# Autodesk Inventor assembly: G20
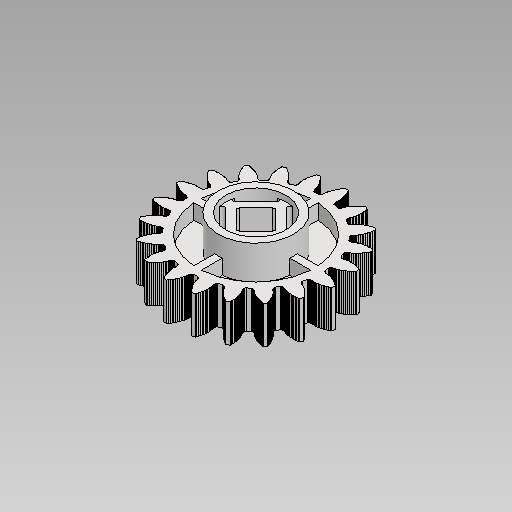
[picture p0: Inventor's stored thumbnail of the model, 512x512]
Saved by Autodesk Inventor 2020 (Build 240168000, 168)
## iProperties
Created: 2019-05-06
Part Number: G20
Document SubType Name: Assembly
Designer: Varga Daniel
Author: Varga Daniel
## Documents named in this file (3)
- C:\!_Dani\!_cloud\OneDrive\!_munka\Revolution\StructuralParts\Gears\G20.iam
- C:\!_Dani\!_cloud\OneDrive\!_munka\Revolution\StructuralParts\Gears\Gear central 20.ipt
- C:\!_Dani\!_cloud\OneDrive\!_munka\Revolution\StructuralParts\Gears\gear20_tooth.ipt
## Components (2 placed, 2 different names)
1. Gear central 20:1 — Mate:1, Mate:2, Mate:3
2. gear20_tooth:1 — Mate:1, Mate:2, Mate:3
## Relationships (3: Mate 3)
- Mate:1: Gear central 20:1 ↔ gear20_tooth:1
- Mate:2: Gear central 20:1 ↔ gear20_tooth:1
- Mate:3: Gear central 20:1 ↔ gear20_tooth:1
